# Autodesk Inventor assembly: robot
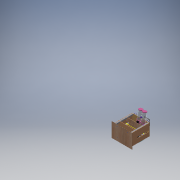
[picture p0: Inventor's stored thumbnail of the model, 180x180]
Saved by Autodesk Inventor 2017 (Build 210142000, 142)
## iProperties
Created: 2018-04-01
Part Number: robot
Document SubType Name: Assembly
Designer: franc
Mass: 1235.72 g
Surface Area: 6399.52 cm^2
Volume: 1204.8 cm^3
Density: 1.02566 g/cm^3
Author: franc
## Documents named in this file (33)
- C:\Users\franc\Desktop\EsialRobotik\Mecanique\2018\robot\robot.iam
- C:\Users\franc\Desktop\EsialRobotik\Mecanique\base_roulante\baseRoulante.iam
- C:\Users\franc\Desktop\EsialRobotik\Mecanique\2018\robot\socle-robot.ipt
- C:\Users\franc\Desktop\EsialRobotik\Mecanique\2018\robot\profile_alu.ipt
- C:\Users\franc\Desktop\EsialRobotik\Mecanique\2018\robot\abeille\lanceur-abeille.iam
- C:\Users\franc\Desktop\EsialRobotik\Mecanique\2018\robot\face-lateral.ipt
- C:\Users\franc\Desktop\EsialRobotik\Mecanique\2018\robot\abeille\lanceur-abeille 2.iam
- C:\Users\franc\Desktop\EsialRobotik\Mecanique\2018\robot\support_arriere.iam
- C:\Users\franc\Desktop\EsialRobotik\Mecanique\2018\robot\toit.ipt
- C:\Users\franc\Desktop\EsialRobotik\Mecanique\composants\SRF04\SRF04_sur_support.iam
- C:\Users\franc\Desktop\EsialRobotik\Mecanique\composants\Interrupteur\arret-urgence.ipt
- C:\Users\franc\Desktop\EsialRobotik\Mecanique\composants\RPlidar-A2M4\RPLIDAR A2.iam
- C:\Users\franc\Desktop\EsialRobotik\Mecanique\composants\Balises\support-balise.ipt
- C:\Users\franc\Desktop\EsialRobotik\Mecanique\composants\Balises\support-lidar.ipt
- C:\Users\franc\Desktop\EsialRobotik\Mecanique\composants\Balises\tige-filletee.ipt
- C:\Users\franc\Desktop\EsialRobotik\Mecanique\composants\Balises\cylindre-mat.ipt
- C:\Users\franc\Desktop\EsialRobotik\Mecanique\2018\robot\traitement-eau\accrocheCremaillereAx12.ipt
- C:\Users\franc\Desktop\EsialRobotik\Mecanique\2018\robot\traitement-eau\accrocheTubesAx12.ipt
- C:\Users\franc\Desktop\EsialRobotik\Mecanique\2018\robot\traitement-eau\cremaillere.ipt
- C:\Users\franc\Desktop\EsialRobotik\Mecanique\2018\robot\traitement-eau\rail.ipt
- C:\Users\franc\Desktop\EsialRobotik\Mecanique\2018\robot\traitement-eau\roueEngrenage.ipt
- C:\Users\franc\Desktop\EsialRobotik\Mecanique\composants\AX12\AX12.iam
- C:\Users\franc\Desktop\EsialRobotik\Mecanique\2018\robot\traitement-eau\cylindre-stockage.ipt
- C:\Users\franc\Desktop\EsialRobotik\Mecanique\2018\robot\etage-bras.ipt
- C:\Users\franc\Desktop\EsialRobotik\Mecanique\2018\robot\traitement-eau\lanceur.iam
- C:\Users\franc\Desktop\EsialRobotik\Mecanique\2018\robot\traitement-eau\bouchon.ipt
- C:\Users\franc\Desktop\EsialRobotik\Mecanique\2018\robot\traitement-eau\support-lanceur.ipt
- C:\Users\franc\Desktop\EsialRobotik\Mecanique\composants\Profile\equerreEtage.ipt
- C:\Users\franc\Desktop\EsialRobotik\Mecanique\2018\robot\etage-carte.ipt
- C:\Users\franc\Desktop\EsialRobotik\Mecanique\2018\robot\traitement-eau\rampe-goulotte.ipt
- C:\Users\franc\Desktop\EsialRobotik\Mecanique\2018\robot\traitement-eau\goulotte.ipt
- C:\Users\franc\Desktop\EsialRobotik\Mecanique\composants\Profile\patin-teflon-24x5.ipt
- C:\Users\franc\Desktop\EsialRobotik\Mecanique\composants\Profile\calle-patin.ipt
## Components (52 placed, 32 different names)
1. baseRoulante:1 [sub-assembly] — Affleurement:1, Affleurement:2, Placage:1, Affleurement:6, Affleurement:7, Affleurement:9, Affleurement:10, Affleurement:12, Placage:34, Placage:66, Affleurement:31, Affleurement:32, Mate:94, Mate:96, Mate:97, Angle:4, Mate:119
2. socle-robot:1 — Affleurement:1, Affleurement:2, Placage:1, Affleurement:5, Affleurement:8, Placage:28, Placage:30, Affleurement:11, Placage:31, Placage:33, Affleurement:13, Placage:35, Affleurement:15, Placage:39, Flush:35, Flush:36, Mate:100, Placage:133, Affleurement:48, Affleurement:49, Placage:135, Affleurement:50, Affleurement:51, Placage:138, Placage:139, Affleurement:52, Affleurement:53, Affleurement:54, Affleurement:55
3. support_arriere:1 [sub-assembly] — Placage:43, Affleurement:16, Flush:38
4. etage-bras:1 — Mate:98, Mate:99, Mate:100, Mate:101, Mate:111, Mate:112, Flush:38, Mate:126, Flush:43, Flush:46
5. etage-carte:1 — Mate:119, Flush:41, Flush:42
6. rampe-goulotte:1 — Mate:126, Flush:43, Mate:127, Flush:45, Flush:46, Flush:47
7. goulotte:1 — Mate:127, Flush:45, Flush:47
8. patin-teflon-24x5:1 — Placage:132, Tangente:5, Tangente:6
9. patin-teflon-24x5:2 — Placage:136, Tangente:9, Tangente:10
10. patin-teflon-24x5:3 — Placage:137, Tangente:11, Tangente:12
11. patin-teflon-24x5:4 — Placage:134, Tangente:7, Tangente:8
12. calle-patin:1 — Placage:134, Placage:135, Tangente:7, Tangente:8, Affleurement:50, Affleurement:51
13. calle-patin:2 — Placage:132, Tangente:5, Tangente:6, Placage:133, Affleurement:48, Affleurement:49
14. calle-patin:3 — Placage:136, Placage:139, Tangente:9, Tangente:10, Affleurement:52, Affleurement:53
15. calle-patin:4 — Placage:137, Placage:138, Tangente:11, Tangente:12, Affleurement:54, Affleurement:55
16. arret-urgence:1 — Placage:53, Tangent:3, Tangent:4
17. SRF04_sur_support:1 [sub-assembly] — Affleurement:23, Placage:49, Mate:103
18. SRF04_sur_support:2 [sub-assembly] — Affleurement:20, Placage:52, Mate:104
19. SRF04_sur_support:3 [sub-assembly] — Affleurement:21, Placage:51, Mate:105
20. SRF04_sur_support:4 [sub-assembly] — Affleurement:22, Placage:50, Mate:106
21. toit:1 — Placage:44, Affleurement:18, Affleurement:19, Affleurement:20, Affleurement:21, Affleurement:22, Affleurement:23, Placage:49, Placage:50, Placage:51, Placage:52, Placage:53, Affleurement:24, Affleurement:25, Tangent:3, Tangent:4, Mate:103, Mate:104, Mate:105, Mate:106, Mate:115, Flush:39, Flush:40, Mate:117
22. lanceur-abeille 2:1 [sub-assembly] — Placage:42, Mate:124, Mate:125
23. lanceur-abeille:1 [sub-assembly] — Placage:36, Mate:122, Mate:123
24. profile_alu:1 — Affleurement:7, Affleurement:8, Placage:28, Placage:43, Mate:99, Flush:41, Flush:42
25. profile_alu:2 — Affleurement:9, Placage:30, Placage:38, Flush:36
26. profile_alu:3 — Affleurement:12, Placage:33, Flush:35
27. profile_alu:4 — Affleurement:10, Affleurement:11, Placage:31
28. face-lateral:1 — Placage:34, Affleurement:13, Placage:35, Placage:36, Affleurement:16, Placage:44, Affleurement:18, Affleurement:19, Mate:122, Mate:123
29. face-lateral:2 — Placage:38, Affleurement:15, Placage:39, Placage:42, Flush:34, Mate:98, Mate:124, Mate:125
30. cylindre-mat:1 — Placage:68, Tangente:1, Tangente:2
31. RPLIDAR A2:1 [sub-assembly] — Placage:54, Placage:55, Placage:56
32. support-balise:1 — Placage:61, Placage:62, Placage:63, Placage:68, Tangente:1, Tangente:2
33. support-lidar:1 — Placage:54, Placage:55, Placage:56, Placage:57, Placage:58, Placage:59, Placage:60, Placage:61, Placage:66, Affleurement:30, Placage:67
34. tige-filletee:1 — Placage:60, Placage:62, Affleurement:28
35. tige-filletee:2 — Placage:59, Affleurement:26, Placage:64
36. tige-filletee:3 — Placage:58, Placage:63, Affleurement:29
37. tige-filletee:4 — Placage:57, Placage:65, Affleurement:27
38. support-balise:2 — Affleurement:26, Placage:64, Placage:65, Affleurement:27, Affleurement:28, Affleurement:29, Affleurement:31
39. equerreEtage:1 — Mate:116, Mate:117, Mate:118
40. support-lanceur:1 — Mate:113, Mate:114, Mate:115, Flush:39, Flush:40, Mate:116, Mate:118
41. bouchon:2 — Mate:109, Mate:110
42. bouchon:1 — Mate:107, Mate:108
43. lanceur:1 [sub-assembly] — Mate:113, Mate:114
44. cylindre-stockage:2 — Mate:88, Mate:90, Angle:3, Mate:109, Mate:110
45. cylindre-stockage:1 — Mate:91, Mate:92, Angle:2, Mate:107, Mate:108
46. accrocheCremaillereAx12:1 — Mate:72, Mate:73, Mate:74, Mate:75, Mate:76, Mate:77
47. accrocheTubesAx12:1 — Mate:78, Mate:79, Mate:80, Mate:88, Mate:90, Mate:91, Mate:92, Angle:2, Angle:3
48. cremaillere:1 — Mate:69, Mate:70, Mate:71, Mate:72, Mate:73, Mate:74, Flush:33
49. rail:1 — Mate:69, Mate:70, Mate:71, Mate:81, Mate:82, Mate:83, Flush:33, Flush:34, Angle:4, Mate:101, Mate:111, Mate:112
50. roueEngrenage:1 — Mate:84, Mate:85, Mate:86
51. AX12:1 [sub-assembly] — Mate:75, Mate:76, Mate:77, Mate:78, Mate:79, Mate:80
52. AX12:2 [sub-assembly] — Mate:81, Mate:82, Mate:83, Mate:84, Mate:85, Mate:86
## Relationships (157: Mate 93, Flush 49, Tangent 12, Angle 3)
- Affleurement:1 [Flush] (5 mm): baseRoulante:1 ↔ socle-robot:1
- Affleurement:2 [Flush] (54 mm): baseRoulante:1 ↔ socle-robot:1
- Placage:1 [Mate]: baseRoulante:1 ↔ socle-robot:1
- Affleurement:5 [Flush]: socle-robot:1
- Affleurement:6 [Flush] (340 mm): baseRoulante:1
- Affleurement:7 [Flush]: baseRoulante:1 ↔ profile_alu:1
- Affleurement:8 [Flush]: socle-robot:1 ↔ profile_alu:1
- Placage:28 [Mate]: socle-robot:1 ↔ profile_alu:1
- Affleurement:9 [Flush]: baseRoulante:1 ↔ profile_alu:2
- Placage:30 [Mate]: socle-robot:1 ↔ profile_alu:2
- Affleurement:10 [Flush]: baseRoulante:1 ↔ profile_alu:4
- Affleurement:11 [Flush]: socle-robot:1 ↔ profile_alu:4
- Placage:31 [Mate]: socle-robot:1 ↔ profile_alu:4
- Affleurement:12 [Flush]: baseRoulante:1 ↔ profile_alu:3
- Placage:33 [Mate]: socle-robot:1 ↔ profile_alu:3
- Placage:34 [Mate]: baseRoulante:1 ↔ face-lateral:1
- Affleurement:13 [Flush]: socle-robot:1 ↔ face-lateral:1
- Placage:35 [Mate]: socle-robot:1 ↔ face-lateral:1
- Placage:36 [Mate]: lanceur-abeille:1 ↔ face-lateral:1
- Placage:38 [Mate]: profile_alu:2 ↔ face-lateral:2
- Affleurement:15 [Flush]: socle-robot:1 ↔ face-lateral:2
- Placage:39 [Mate]: socle-robot:1 ↔ face-lateral:2
- Placage:42 [Mate]: lanceur-abeille 2:1 ↔ face-lateral:2
- Placage:43 [Mate]: support_arriere:1 ↔ profile_alu:1
- Affleurement:16 [Flush]: support_arriere:1 ↔ face-lateral:1
- Placage:44 [Mate]: toit:1 ↔ face-lateral:1
- Affleurement:18 [Flush]: toit:1 ↔ face-lateral:1
- Affleurement:19 [Flush]: toit:1 ↔ face-lateral:1
- Affleurement:20 [Flush]: SRF04_sur_support:2 ↔ toit:1
- Affleurement:21 [Flush]: SRF04_sur_support:3 ↔ toit:1
- Affleurement:22 [Flush]: SRF04_sur_support:4 ↔ toit:1
- Affleurement:23 [Flush]: SRF04_sur_support:1 ↔ toit:1
- Placage:49 [Mate]: SRF04_sur_support:1 ↔ toit:1
- Placage:50 [Mate]: SRF04_sur_support:4 ↔ toit:1
- Placage:51 [Mate]: SRF04_sur_support:3 ↔ toit:1
- Placage:52 [Mate]: SRF04_sur_support:2 ↔ toit:1
- Placage:53 [Mate]: arret-urgence:1 ↔ toit:1
- Affleurement:24 [Flush] (-150 mm): toit:1
- Affleurement:25 [Flush] (-100 mm): toit:1
- Placage:54 [Mate]: RPLIDAR A2:1 ↔ support-lidar:1
- Placage:55 [Mate]: RPLIDAR A2:1 ↔ support-lidar:1
- Placage:56 [Mate]: RPLIDAR A2:1 ↔ support-lidar:1
- Placage:57 [Mate]: support-lidar:1 ↔ tige-filletee:4
- Placage:58 [Mate]: support-lidar:1 ↔ tige-filletee:3
- Placage:59 [Mate]: support-lidar:1 ↔ tige-filletee:2
- Placage:60 [Mate]: support-lidar:1 ↔ tige-filletee:1
- Placage:61 [Mate] (45 mm): support-balise:1 ↔ support-lidar:1
- Placage:62 [Mate]: support-balise:1 ↔ tige-filletee:1
- Placage:63 [Mate]: support-balise:1 ↔ tige-filletee:3
- Affleurement:26 [Flush]: tige-filletee:2 ↔ support-balise:2
- Placage:64 [Mate]: tige-filletee:2 ↔ support-balise:2
- Placage:65 [Mate]: tige-filletee:4 ↔ support-balise:2
- Affleurement:27 [Flush]: tige-filletee:4 ↔ support-balise:2
- Affleurement:28 [Flush]: tige-filletee:1 ↔ support-balise:2
- Affleurement:29 [Flush]: tige-filletee:3 ↔ support-balise:2
- Placage:66 [Mate] (330 mm): baseRoulante:1 ↔ support-lidar:1
- Affleurement:30 [Flush]: support-lidar:1
- Placage:67 [Mate]: support-lidar:1
- Affleurement:31 [Flush] (-430 mm): baseRoulante:1 ↔ support-balise:2
- Affleurement:32 [Flush] (350 mm): baseRoulante:1
- Placage:68 [Mate]: cylindre-mat:1 ↔ support-balise:1
- Tangente:1: cylindre-mat:1 ↔ support-balise:1
- Tangente:2: cylindre-mat:1 ↔ support-balise:1
- Mate:69: cremaillere:1 ↔ rail:1
- Mate:70: cremaillere:1 ↔ rail:1
- Mate:71: cremaillere:1 ↔ rail:1
- Mate:72: accrocheCremaillereAx12:1 ↔ cremaillere:1
- Mate:73: accrocheCremaillereAx12:1 ↔ cremaillere:1
- Mate:74: accrocheCremaillereAx12:1 ↔ cremaillere:1
- Mate:75: accrocheCremaillereAx12:1 ↔ AX12:1
- Mate:76: accrocheCremaillereAx12:1 ↔ AX12:1
- Mate:77: accrocheCremaillereAx12:1 ↔ AX12:1
- Mate:78: accrocheTubesAx12:1 ↔ AX12:1
- Mate:79: accrocheTubesAx12:1 ↔ AX12:1
- Mate:80: accrocheTubesAx12:1 ↔ AX12:1
- Mate:81: rail:1 ↔ AX12:2
- Mate:82: rail:1 ↔ AX12:2
- Mate:83: rail:1 ↔ AX12:2
- Mate:84: roueEngrenage:1 ↔ AX12:2
- Mate:85: roueEngrenage:1 ↔ AX12:2
- Mate:86: roueEngrenage:1 ↔ AX12:2
- Mate:88: cylindre-stockage:2 ↔ accrocheTubesAx12:1
- Mate:90: cylindre-stockage:2 ↔ accrocheTubesAx12:1
- Mate:91: cylindre-stockage:1 ↔ accrocheTubesAx12:1
- Mate:92: cylindre-stockage:1 ↔ accrocheTubesAx12:1
- Angle:2 (0 deg): cylindre-stockage:1 ↔ accrocheTubesAx12:1
- Angle:3 (0 deg): cylindre-stockage:2 ↔ accrocheTubesAx12:1
- Mate:94: baseRoulante:1
- Tangent:3 (30 mm): arret-urgence:1 ↔ toit:1
- Tangent:4 (30 mm): arret-urgence:1 ↔ toit:1
- Mate:96 (-125 mm): baseRoulante:1
- Mate:97 (175 mm): baseRoulante:1
- Flush:33 (-45 mm): cremaillere:1 ↔ rail:1
- Flush:34 (70 mm): face-lateral:2 ↔ rail:1
- Angle:4 (180 deg): baseRoulante:1 ↔ rail:1
- Flush:35: socle-robot:1 ↔ profile_alu:3
- Flush:36: socle-robot:1 ↔ profile_alu:2
- Mate:98: etage-bras:1 ↔ face-lateral:2
- Mate:99: etage-bras:1 ↔ profile_alu:1
- Mate:100 (192 mm): socle-robot:1 ↔ etage-bras:1
- Mate:101: etage-bras:1 ↔ rail:1
- Mate:103: SRF04_sur_support:1 ↔ toit:1
- Mate:104: SRF04_sur_support:2 ↔ toit:1
- Mate:105: SRF04_sur_support:3 ↔ toit:1
- Mate:106: SRF04_sur_support:4 ↔ toit:1
- Mate:107: bouchon:1 ↔ cylindre-stockage:1
- Mate:108: bouchon:1 ↔ cylindre-stockage:1
- Mate:109: bouchon:2 ↔ cylindre-stockage:2
- Mate:110: bouchon:2 ↔ cylindre-stockage:2
- Mate:111: etage-bras:1 ↔ rail:1
- Mate:112: etage-bras:1 ↔ rail:1
- Mate:113: support-lanceur:1 ↔ lanceur:1
- Mate:114: support-lanceur:1 ↔ lanceur:1
- Mate:115: toit:1 ↔ support-lanceur:1
- Flush:38: support_arriere:1 ↔ etage-bras:1
- Flush:39 (35 mm): toit:1 ↔ support-lanceur:1
- Flush:40 (55 mm): toit:1 ↔ support-lanceur:1
- Mate:116: equerreEtage:1 ↔ support-lanceur:1
- Mate:117: toit:1 ↔ equerreEtage:1
- Mate:118: equerreEtage:1 ↔ support-lanceur:1
- Mate:119 (90 mm): baseRoulante:1 ↔ etage-carte:1
- Flush:41: etage-carte:1 ↔ profile_alu:1
- Flush:42: etage-carte:1 ↔ profile_alu:1
- Mate:122: lanceur-abeille:1 ↔ face-lateral:1
- Mate:123: lanceur-abeille:1 ↔ face-lateral:1
- Mate:124: lanceur-abeille 2:1 ↔ face-lateral:2
- Mate:125: lanceur-abeille 2:1 ↔ face-lateral:2
- Mate:126: etage-bras:1 ↔ rampe-goulotte:1
- Flush:43: etage-bras:1 ↔ rampe-goulotte:1
- Mate:127: rampe-goulotte:1 ↔ goulotte:1
- Flush:45: rampe-goulotte:1 ↔ goulotte:1
- Flush:46 (-50 mm): etage-bras:1 ↔ rampe-goulotte:1
- Flush:47 (-22 mm): rampe-goulotte:1 ↔ goulotte:1
- Placage:132 [Mate]: patin-teflon-24x5:1 ↔ calle-patin:2
- Tangente:5 (5 mm): patin-teflon-24x5:1 ↔ calle-patin:2
- Tangente:6 (5 mm): patin-teflon-24x5:1 ↔ calle-patin:2
- Placage:133 [Mate]: socle-robot:1 ↔ calle-patin:2
- Affleurement:48 [Flush]: socle-robot:1 ↔ calle-patin:2
- Affleurement:49 [Flush] (40 mm): socle-robot:1 ↔ calle-patin:2
- Placage:134 [Mate]: patin-teflon-24x5:4 ↔ calle-patin:1
- Placage:135 [Mate]: socle-robot:1 ↔ calle-patin:1
- Tangente:7 (5 mm): patin-teflon-24x5:4 ↔ calle-patin:1
- Tangente:8 (5 mm): patin-teflon-24x5:4 ↔ calle-patin:1
- Affleurement:50 [Flush]: socle-robot:1 ↔ calle-patin:1
- Affleurement:51 [Flush] (40 mm): socle-robot:1 ↔ calle-patin:1
- Placage:136 [Mate]: patin-teflon-24x5:2 ↔ calle-patin:3
- Placage:137 [Mate]: patin-teflon-24x5:3 ↔ calle-patin:4
- Placage:138 [Mate]: socle-robot:1 ↔ calle-patin:4
- Placage:139 [Mate]: socle-robot:1 ↔ calle-patin:3
- Tangente:9 (5 mm): patin-teflon-24x5:2 ↔ calle-patin:3
- Tangente:10 (5 mm): patin-teflon-24x5:2 ↔ calle-patin:3
- Affleurement:52 [Flush] (40 mm): socle-robot:1 ↔ calle-patin:3
- Affleurement:53 [Flush]: socle-robot:1 ↔ calle-patin:3
- Tangente:11 (5 mm): patin-teflon-24x5:3 ↔ calle-patin:4
- Tangente:12 (5 mm): patin-teflon-24x5:3 ↔ calle-patin:4
- Affleurement:54 [Flush] (40 mm): socle-robot:1 ↔ calle-patin:4
- Affleurement:55 [Flush]: socle-robot:1 ↔ calle-patin:4
